# Autodesk Inventor assembly: 5-7
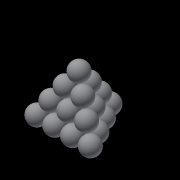
[picture p0: Inventor's stored thumbnail of the model, 180x180]
Saved by Autodesk Inventor 2017 (Build 210142000, 142)
## iProperties
Part Number: 5-7
Material: 一般
Document SubType Name: Assembly
Designer: r0909
Author: r0909
## Documents named in this file (3)
- C:\Users\r0909\Desktop\inventor\5-7.iam
- C:\Users\r0909\Desktop\inventor\5-6b.iam
- C:\Users\r0909\Desktop\inventor\5-6c.iam
## Components (6 placed, 2 different names)
1. 5-6b:1 [sub-assembly] — 齊平:1, 相切:1, 相切:2, 相切:5, 相切:8, 相切:9, 相切:14, 相切:15
2. 5-6c:1 [sub-assembly] — 齊平:1, 相切:1, 相切:2, 相切:3, 相切:4, 相切:6, 相切:7
3. 5-6b:2 [sub-assembly] — 相切:3, 相切:4, 相切:5, 相切:6, 相切:7, 相切:10, 相切:11, 相切:12, 相切:13, 相切:16, 相切:17, 相切:18, 相切:19
4. 5-6b:3 [sub-assembly] — 相切:8, 相切:9, 相切:10, 相切:11, 相切:12, 相切:13, 相切:21, 相切:23, 相切:24, 相切:27
5. 5-6b:4 [sub-assembly] — 相切:14, 相切:15, 相切:16, 相切:17, 相切:18, 相切:19, 相切:20, 相切:22, 相切:25, 相切:26
6. 5-6c:2 [sub-assembly] — 相切:20, 相切:21, 相切:22, 相切:23, 相切:24, 相切:25, 相切:26, 相切:27
## Relationships (28: Tangent 27, Flush 1)
- 齊平:1 [Flush]: 5-6b:1 ↔ 5-6c:1
- 相切:1 [Tangent]: 5-6b:1 ↔ 5-6c:1
- 相切:2 [Tangent]: 5-6b:1 ↔ 5-6c:1
- 相切:3 [Tangent]: 5-6c:1 ↔ 5-6b:2
- 相切:4 [Tangent]: 5-6c:1 ↔ 5-6b:2
- 相切:5 [Tangent]: 5-6b:1 ↔ 5-6b:2
- 相切:6 [Tangent]: 5-6c:1 ↔ 5-6b:2
- 相切:7 [Tangent]: 5-6c:1 ↔ 5-6b:2
- 相切:8 [Tangent]: 5-6b:1 ↔ 5-6b:3
- 相切:9 [Tangent]: 5-6b:1 ↔ 5-6b:3
- 相切:10 [Tangent]: 5-6b:2 ↔ 5-6b:3
- 相切:11 [Tangent]: 5-6b:2 ↔ 5-6b:3
- 相切:12 [Tangent]: 5-6b:2 ↔ 5-6b:3
- 相切:13 [Tangent]: 5-6b:2 ↔ 5-6b:3
- 相切:14 [Tangent]: 5-6b:1 ↔ 5-6b:4
- 相切:15 [Tangent]: 5-6b:1 ↔ 5-6b:4
- 相切:16 [Tangent]: 5-6b:2 ↔ 5-6b:4
- 相切:17 [Tangent]: 5-6b:2 ↔ 5-6b:4
- 相切:18 [Tangent]: 5-6b:2 ↔ 5-6b:4
- 相切:19 [Tangent]: 5-6b:2 ↔ 5-6b:4
- 相切:20 [Tangent]: 5-6b:4 ↔ 5-6c:2
- 相切:21 [Tangent]: 5-6b:3 ↔ 5-6c:2
- 相切:22 [Tangent]: 5-6b:4 ↔ 5-6c:2
- 相切:23 [Tangent]: 5-6b:3 ↔ 5-6c:2
- 相切:24 [Tangent]: 5-6b:3 ↔ 5-6c:2
- 相切:25 [Tangent]: 5-6b:4 ↔ 5-6c:2
- 相切:26 [Tangent]: 5-6b:4 ↔ 5-6c:2
- 相切:27 [Tangent]: 5-6b:3 ↔ 5-6c:2
